# Autodesk Inventor assembly: ExtensionArm
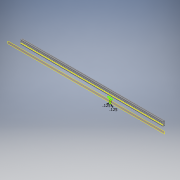
[picture p0: Inventor's stored thumbnail of the model, 180x180]
Saved by Autodesk Inventor 2018 (Build 220112000, 112)
## iProperties
Created: 2017-11-15
Part Number: ExtensionArm
Document SubType Name: Assembly
Designer: ball
Author: ball
## Documents named in this file (3)
- C:\FTC\FTC8863CAD\2017Robot\ExtensionArm.iam
- C:\FTC\FTC8863CAD\Actobotics\605 parts\605630.ipt
- C:\FTC\FTC8863CAD\RevRobotics\REV-41-1017.ipt
## Components (3 placed, 2 different names)
1. 605630:1
2. REV-41-1017:1 — Flush:1, Flush:2, Mate:1, Flush:3
3. REV-41-1017:2 — Flush:1, Flush:2, Mate:1
## Relationships (4: Flush 3, Mate 1)
- Flush:1: REV-41-1017:1 ↔ REV-41-1017:2
- Flush:2: REV-41-1017:1 ↔ REV-41-1017:2
- Mate:1 (2.3368 mm): REV-41-1017:1 ↔ REV-41-1017:2
- Flush:3 (38.1 mm): REV-41-1017:1
